# Autodesk Inventor assembly: ASY MSC 010 cone
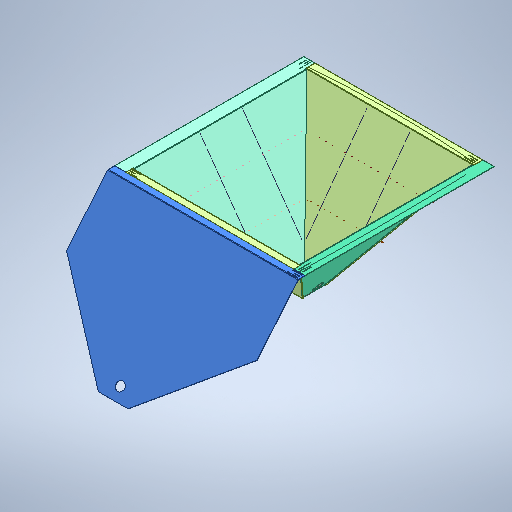
[picture p0: Inventor's stored thumbnail of the model, 512x512]
Saved by Autodesk Inventor 2025 (Build 290162010, 162A)
## iProperties
Created: 2024-05-19
Part Number: ASY MSC 010 cone
Document SubType Name: Assembly
Designer: admin
Mass: 24706.5 g
Surface Area: 124528 cm^2
Volume: 24706.5 cm^3
Density: 1 g/cm^3
Stock Number: ASY МОО 010 конус
Author: admin
## Documents named in this file (13)
- C:\Users\pokla\Documents\Inventor\Отстойник осветлитель\Manturovo_Se-clar-Gleb\ASY MSC 010 cone.iam
- C:\Users\pokla\Documents\Inventor\Отстойник осветлитель\Manturovo_Se-clar-Gleb\конус\MSC 014 cone IN right board.ipt
- C:\Users\pokla\Documents\Inventor\Отстойник осветлитель\Manturovo_Se-clar-Gleb\конус\MSC 011 cone IN bottom.ipt
- C:\Users\pokla\Documents\Inventor\Отстойник осветлитель\Manturovo_Se-clar-Gleb\конус\MSC 013 cone IN left board.ipt
- C:\Users\pokla\Documents\Inventor\Отстойник осветлитель\Manturovo_Se-clar-Gleb\конус\MSC 012 cone IN back.ipt
- C:\Users\pokla\Documents\Inventor\Отстойник осветлитель\Manturovo_Se-clar-Gleb\конус\MSC 019 cone sketch.ipt
- C:\Users\pokla\Documents\Inventor\Отстойник осветлитель\Manturovo_Se-clar-Gleb\конус\MSC 015 cone IN bow.ipt
- C:\Users\pokla\Documents\Inventor\Отстойник осветлитель\Manturovo_Se-clar-Gleb\конус\MSC 016 cone exit back.ipt
- C:\Users\pokla\Documents\Inventor\Отстойник осветлитель\Manturovo_Se-clar-Gleb\DXF файлы\MSC 0691 stringer cone.ipt
- C:\Users\pokla\Documents\Inventor\Отстойник осветлитель\Manturovo_Se-clar-Gleb\DXF файлы\MSC 0561 rib cone.ipt
- C:\Users\pokla\Documents\Inventor\Отстойник осветлитель\Manturovo_Se-clar-Gleb\DXF файлы\MSC 0562 rib cone.ipt
- C:\Users\pokla\Documents\Inventor\Отстойник осветлитель\Manturovo_Se-clar-Gleb\DXF файлы\MSC 0563 rib cone.ipt
- C:\Users\pokla\Documents\Inventor\Отстойник осветлитель\Manturovo_Se-clar-Gleb\DXF файлы\MSC 0564 rib cone.ipt
## Components (15 placed, 12 different names)
1. MSC 019 cone sketch.ipt:1 — Flush:8, Flush:9, Mate:1
2. MSC 012 cone IN back.ipt:1 — Flush:6, Flush:10, Mate:2, Flush:12, Mate:23, Mate:27, Mate:32, Mate:33, Mate:38
3. MSC 011 cone IN bottom.ipt:1 — Flush:4, Flush:5, Flush:11, Flush:21
4. MSC 014 cone IN right board.ipt:1 — Flush:12, Flush:13, Flush:15, Mate:28, Mate:37, Mate:39
5. MSC 013 cone IN left board.ipt:1 — Mate:4, Flush:14, Mate:5
6. MSC 015 cone IN bow.ipt:1 — Mate:3, Mate:6, Flush:16, Flush:17, Rigid:1
7. MSC 016 cone exit back.ipt:1 — Rigid:1
8. MSC 0562 rib cone:1 — Mate:27, Mate:30, Mate:31
9. MSC 0561 rib cone:1 — Mate:32, Mate:33, Mate:34
10. MSC 0691 stringer cone:1 — Mate:23, Rigid:2, Mate:41
11. MSC 0564 rib cone:1 — Mate:46, Mate:47
12. MSC 0563 rib cone:1 — Mate:37, Mate:45, Mate:48
13. MSC 0691 stringer cone:2 — Mate:38, Mate:39, Mate:40, Mate:42, Mate:43, Flush:22
14. MSC 0691 stringer cone:3 — Rigid:2, Mate:30, Mate:31, Mate:34
15. MSC 0691 stringer cone:4 — Mate:28, Mate:43, Flush:22, Mate:45, Mate:46, Mate:47, Mate:48
## Relationships (44: Mate 26, Flush 16, WeldJoint 2)
- Flush:4: MSC 011 cone IN bottom.ipt:1
- Flush:5: MSC 011 cone IN bottom.ipt:1
- Flush:6: MSC 012 cone IN back.ipt:1
- Flush:8: MSC 019 cone sketch.ipt:1
- Flush:9: MSC 019 cone sketch.ipt:1
- Mate:1: MSC 019 cone sketch.ipt:1
- Flush:10: MSC 012 cone IN back.ipt:1
- Mate:2: MSC 012 cone IN back.ipt:1
- Flush:11 (-230 mm): MSC 011 cone IN bottom.ipt:1
- Mate:3: MSC 015 cone IN bow.ipt:1
- Flush:12: MSC 012 cone IN back.ipt:1 ↔ MSC 014 cone IN right board.ipt:1
- Flush:13: MSC 014 cone IN right board.ipt:1
- Mate:4: MSC 013 cone IN left board.ipt:1
- Flush:14: MSC 013 cone IN left board.ipt:1
- Mate:5: MSC 013 cone IN left board.ipt:1
- Flush:15: MSC 014 cone IN right board.ipt:1
- Mate:6: MSC 015 cone IN bow.ipt:1
- Flush:16: MSC 015 cone IN bow.ipt:1
- Flush:17: MSC 015 cone IN bow.ipt:1
- Rigid:1 [WeldJoint]: MSC 015 cone IN bow.ipt:1 ↔ MSC 016 cone exit back.ipt:1
- [Mate]: MSC 0562 rib cone:1
- [Flush]: MSC 014 cone IN right board.ipt:1 ↔ MSC 0564 rib cone:1
- Mate:23: MSC 012 cone IN back.ipt:1 ↔ MSC 0691 stringer cone:1
- Rigid:2 [WeldJoint] (377 mm): MSC 0691 stringer cone:1 ↔ MSC 0691 stringer cone:3
- Mate:27: MSC 012 cone IN back.ipt:1 ↔ MSC 0562 rib cone:1
- Mate:28: MSC 014 cone IN right board.ipt:1 ↔ MSC 0691 stringer cone:4
- Mate:30: MSC 0562 rib cone:1 ↔ MSC 0691 stringer cone:3
- Mate:31: MSC 0562 rib cone:1 ↔ MSC 0691 stringer cone:3
- Mate:32: MSC 012 cone IN back.ipt:1 ↔ MSC 0561 rib cone:1
- Mate:33: MSC 012 cone IN back.ipt:1 ↔ MSC 0561 rib cone:1
- Mate:34: MSC 0561 rib cone:1 ↔ MSC 0691 stringer cone:3
- Mate:37: MSC 014 cone IN right board.ipt:1 ↔ MSC 0563 rib cone:1
- Mate:38 (188.5 mm): MSC 012 cone IN back.ipt:1 ↔ MSC 0691 stringer cone:2
- Mate:39: MSC 014 cone IN right board.ipt:1 ↔ MSC 0691 stringer cone:2
- Flush:21 (-160 mm): MSC 011 cone IN bottom.ipt:1
- Mate:40: MSC 0691 stringer cone:2
- Mate:41: MSC 0691 stringer cone:1
- Mate:42: MSC 0691 stringer cone:2
- Mate:43 (377 mm): MSC 0691 stringer cone:2 ↔ MSC 0691 stringer cone:4
- Flush:22: MSC 0691 stringer cone:2 ↔ MSC 0691 stringer cone:4
- Mate:45: MSC 0563 rib cone:1 ↔ MSC 0691 stringer cone:4
- Mate:46 (2 mm): MSC 0564 rib cone:1 ↔ MSC 0691 stringer cone:4
- Mate:47: MSC 0564 rib cone:1 ↔ MSC 0691 stringer cone:4
- Mate:48 (2 mm): MSC 0563 rib cone:1 ↔ MSC 0691 stringer cone:4
